# Autodesk Inventor assembly: Jar Jar
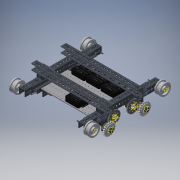
[picture p0: Inventor's stored thumbnail of the model, 180x180]
Saved by Autodesk Inventor 2016 (Build 200138000, 138)
## iProperties
Created: 2015-12-13
Part Number: Jar Jar
Document SubType Name: Assembly
Designer: tbloo
Author: tbloo
## Documents named in this file (16)
- C:\Users\tbloo\Documents\GitHub\phi_robotics\3d-models\FTC_Tetrix_KOP_Block_Party\Tim Bloot Designs\JAr JaR Bot\Jar Jar.iam
- C:\Users\tbloo\Documents\GitHub\phi_robotics\3d-models\FTC_Tetrix_KOP_Block_Party\Tim Bloot Designs\Base Plate.ipt
- C:\Users\tbloo\Documents\GitHub\phi_robotics\3d-models\FTC_Tetrix_KOP_Block_Party\Tetrix_Kit_FTC\Autodesk Inventor Files\tetrix_c_channel-3.ipt
- C:\Users\tbloo\Documents\GitHub\phi_robotics\3d-models\FTC_Tetrix_KOP_Block_Party\Tetrix_Kit_FTC\Autodesk Inventor Files\tetrix_c_channel-2.ipt
- C:\Users\tbloo\Documents\GitHub\phi_robotics\3d-models\FTC_Tetrix_KOP_Block_Party\Tetrix_Kit_FTC\Autodesk Inventor Files\tetrix_motor_mount-old.ipt
- C:\Users\tbloo\Documents\GitHub\phi_robotics\3d-models\FTC_Tetrix_KOP_Block_Party\Tetrix_Kit_FTC\Autodesk Inventor Files\tetrix_739274_2013.ipt
- C:\Users\tbloo\Documents\GitHub\phi_robotics\3d-models\FTC_Tetrix_KOP_Block_Party\Tetrix_Kit_FTC\Autodesk Inventor Files\tetrix_motor.iam
- C:\Users\tbloo\Documents\GitHub\phi_robotics\3d-models\FTC_Tetrix_KOP_Block_Party\Tim Bloot Designs\JAr JaR Bot\Motor Med Gear.iam
- C:\Users\tbloo\Documents\GitHub\phi_robotics\3d-models\FTC_Tetrix_KOP_Block_Party\Tim Bloot Designs\JAr JaR Bot\Tread Sproket Gear Assembly.iam
- C:\Users\tbloo\Documents\GitHub\phi_robotics\3d-models\FTC_Tetrix_KOP_Block_Party\Tetrix_Kit_FTC\Autodesk Inventor Files\tetrix_bushing.ipt
- C:\Users\tbloo\Documents\GitHub\phi_robotics\3d-models\FTC_Tetrix_KOP_Block_Party\Tim Bloot Designs\JAr JaR Bot\Tread Wheel Assembly.iam
- C:\Users\tbloo\Documents\GitHub\phi_robotics\3d-models\FTC_Tetrix_KOP_Block_Party\Tetrix_Kit_FTC\Autodesk Inventor Files\tetrix_angle-144 MM.ipt
- C:\Users\tbloo\Documents\GitHub\phi_robotics\3d-models\FTC_Tetrix_KOP_Block_Party\Tetrix_Kit_FTC\Autodesk Inventor Files\tetrix_c_channel-5.ipt
- C:\Users\tbloo\Documents\GitHub\phi_robotics\3d-models\FTC_Tetrix_KOP_Block_Party\Tetrix_Kit_FTC\Autodesk Inventor Files\tetrix_inside_corner_bracket.ipt
- C:\Users\tbloo\Documents\GitHub\phi_robotics\3d-models\FTC_Tetrix_KOP_Block_Party\Tetrix_Kit_FTC\Autodesk Inventor Files\tetrix_motor_controller.ipt
- C:\Users\tbloo\Documents\GitHub\phi_robotics\3d-models\FTC_Tetrix_KOP_Block_Party\Tetrix_Kit_FTC\Autodesk Inventor Files\tetrix_servo_controller.ipt
## Components (55 placed, 15 different names)
1. Base Plate:1 — Rigid:40, Rigid:53, Rigid:60, Rigid:61, Rigid:63
2. tetrix_c_channel-3:3 — Rigid:37, Rigid:39, Rigid:54, Rigid:57
3. tetrix_c_channel-2:9
4. tetrix_c_channel-2:10
5. tetrix_c_channel-2:11 — Rigid:38
6. tetrix_c_channel-2:12 — Rigid:36
7. tetrix_motor_mount-old:3
8. tetrix_motor_mount-old:4
9. tetrix_739274_2013:3
10. tetrix_739274_2013:4
11. tetrix_motor:3 [sub-assembly]
12. tetrix_motor:4 [sub-assembly]
13. Motor Med Gear:3 [sub-assembly]
14. Motor Med Gear:4 [sub-assembly]
15. Tread Sproket Gear Assembly:3 [sub-assembly]
16. Tread Sproket Gear Assembly:4 [sub-assembly]
17. tetrix_bushing:5
18. tetrix_bushing:6
19. tetrix_bushing:7
20. tetrix_bushing:8
21. Tread Wheel Assembly:3 [sub-assembly]
22. Tread Wheel Assembly:4 [sub-assembly]
23. tetrix_angle-144 MM:1 — Rigid:36, Rigid:37, Rigid:40
24. tetrix_angle-144 MM:2 — Rigid:38, Rigid:39
25. tetrix_c_channel-3:4 — Rigid:55, Rigid:56
26. tetrix_c_channel-2:13
27. tetrix_c_channel-2:14
28. tetrix_c_channel-2:15
29. tetrix_c_channel-2:16
30. tetrix_motor_mount-old:5
31. tetrix_motor_mount-old:6
32. tetrix_739274_2013:5
33. tetrix_739274_2013:6
34. tetrix_motor:5 [sub-assembly]
35. tetrix_motor:6 [sub-assembly]
36. Motor Med Gear:5 [sub-assembly]
37. Motor Med Gear:6 [sub-assembly]
38. Tread Sproket Gear Assembly:5 [sub-assembly]
39. Tread Sproket Gear Assembly:6 [sub-assembly]
40. tetrix_bushing:9
41. tetrix_bushing:10
42. tetrix_bushing:11
43. tetrix_bushing:12
44. Tread Wheel Assembly:5 [sub-assembly]
45. Tread Wheel Assembly:6 [sub-assembly]
46. tetrix_angle-144 MM:3
47. tetrix_angle-144 MM:4 — Rigid:53
48. tetrix_c_channel-5:1 — Rigid:54, Rigid:55
49. tetrix_c_channel-5:2 — Rigid:58, Rigid:59
50. tetrix_inside_corner_bracket:1 — Rigid:57, Rigid:58
51. tetrix_inside_corner_bracket:2 — Rigid:56, Rigid:59
52. tetrix_motor_controller:1 — Rigid:61, Rigid:62
53. tetrix_motor_controller:2 — Rigid:60
54. tetrix_motor_controller:3 — Rigid:62
55. tetrix_servo_controller:1 — Rigid:63
## Relationships (56: WeldJoint 36, RevoluteJoint 20)
- [WeldJoint]: tetrix_c_channel-2:9 ↔ tetrix_motor_mount-old:4
- [WeldJoint]: tetrix_c_channel-2:10 ↔ tetrix_motor_mount-old:3
- [WeldJoint]: tetrix_c_channel-2:9 ↔ tetrix_739274_2013:3
- [WeldJoint]: tetrix_c_channel-2:11 ↔ tetrix_739274_2013:3
- [WeldJoint]: tetrix_c_channel-2:10 ↔ tetrix_739274_2013:4
- [WeldJoint]: tetrix_c_channel-2:12 ↔ tetrix_739274_2013:4
- [RevoluteJoint]: tetrix_motor_mount-old:4 ↔ tetrix_motor:3
- [RevoluteJoint]: tetrix_motor_mount-old:3 ↔ tetrix_motor:4
- [WeldJoint] (-7.5 mm): tetrix_motor:4 ↔ Motor Med Gear:3
- [WeldJoint] (-7.5 mm): tetrix_motor:3 ↔ Motor Med Gear:4
- [RevoluteJoint]: tetrix_c_channel-2:9 ↔ tetrix_bushing:6
- [RevoluteJoint]: tetrix_c_channel-2:9 ↔ tetrix_bushing:5
- [RevoluteJoint]: Tread Sproket Gear Assembly:3 ↔ tetrix_bushing:5
- [RevoluteJoint]: tetrix_c_channel-2:10 ↔ tetrix_bushing:7
- [RevoluteJoint]: tetrix_c_channel-2:10 ↔ tetrix_bushing:8
- [RevoluteJoint]: Tread Sproket Gear Assembly:4 ↔ tetrix_bushing:8
- [RevoluteJoint]: tetrix_c_channel-2:11 ↔ Tread Wheel Assembly:3
- [RevoluteJoint]: tetrix_c_channel-2:12 ↔ Tread Wheel Assembly:4
- Rigid:36 [WeldJoint]: tetrix_c_channel-2:12 ↔ tetrix_angle-144 MM:1
- Rigid:37 [WeldJoint]: tetrix_c_channel-3:3 ↔ tetrix_angle-144 MM:1
- Rigid:38 [WeldJoint]: tetrix_c_channel-2:11 ↔ tetrix_angle-144 MM:2
- Rigid:39 [WeldJoint]: tetrix_c_channel-3:3 ↔ tetrix_angle-144 MM:2
- Rigid:40 [WeldJoint]: Base Plate:1 ↔ tetrix_angle-144 MM:1
- [WeldJoint]: tetrix_c_channel-2:13 ↔ tetrix_motor_mount-old:6
- [WeldJoint]: tetrix_c_channel-2:14 ↔ tetrix_motor_mount-old:5
- [WeldJoint]: tetrix_c_channel-2:13 ↔ tetrix_739274_2013:5
- [WeldJoint]: tetrix_c_channel-2:15 ↔ tetrix_739274_2013:5
- [WeldJoint]: tetrix_c_channel-2:14 ↔ tetrix_739274_2013:6
- [WeldJoint]: tetrix_c_channel-2:16 ↔ tetrix_739274_2013:6
- [RevoluteJoint]: tetrix_motor_mount-old:6 ↔ tetrix_motor:5
- [RevoluteJoint]: tetrix_motor_mount-old:5 ↔ tetrix_motor:6
- [WeldJoint] (-7.5 mm): tetrix_motor:6 ↔ Motor Med Gear:5
- [WeldJoint] (-7.5 mm): tetrix_motor:5 ↔ Motor Med Gear:6
- [RevoluteJoint]: tetrix_c_channel-2:13 ↔ tetrix_bushing:10
- [RevoluteJoint]: tetrix_c_channel-2:13 ↔ tetrix_bushing:9
- [RevoluteJoint]: Tread Sproket Gear Assembly:5 ↔ tetrix_bushing:9
- [RevoluteJoint]: tetrix_c_channel-2:14 ↔ tetrix_bushing:11
- [RevoluteJoint]: tetrix_c_channel-2:14 ↔ tetrix_bushing:12
- [RevoluteJoint]: Tread Sproket Gear Assembly:6 ↔ tetrix_bushing:12
- [RevoluteJoint]: tetrix_c_channel-2:15 ↔ Tread Wheel Assembly:5
- [RevoluteJoint]: tetrix_c_channel-2:16 ↔ Tread Wheel Assembly:6
- [WeldJoint]: tetrix_c_channel-2:16 ↔ tetrix_angle-144 MM:3
- [WeldJoint]: tetrix_c_channel-3:4 ↔ tetrix_angle-144 MM:3
- [WeldJoint]: tetrix_c_channel-2:15 ↔ tetrix_angle-144 MM:4
- [WeldJoint]: tetrix_c_channel-3:4 ↔ tetrix_angle-144 MM:4
- Rigid:53 [WeldJoint]: Base Plate:1 ↔ tetrix_angle-144 MM:4
- Rigid:54 [WeldJoint]: tetrix_c_channel-3:3 ↔ tetrix_c_channel-5:1
- Rigid:55 [WeldJoint]: tetrix_c_channel-3:4 ↔ tetrix_c_channel-5:1
- Rigid:56 [WeldJoint]: tetrix_c_channel-3:4 ↔ tetrix_inside_corner_bracket:2
- Rigid:57 [WeldJoint]: tetrix_c_channel-3:3 ↔ tetrix_inside_corner_bracket:1
- Rigid:58 [WeldJoint]: tetrix_c_channel-5:2 ↔ tetrix_inside_corner_bracket:1
- Rigid:59 [WeldJoint]: tetrix_c_channel-5:2 ↔ tetrix_inside_corner_bracket:2
- Rigid:60 [WeldJoint]: Base Plate:1 ↔ tetrix_motor_controller:2
- Rigid:61 [WeldJoint]: Base Plate:1 ↔ tetrix_motor_controller:1
- Rigid:62 [WeldJoint]: tetrix_motor_controller:1 ↔ tetrix_motor_controller:3
- Rigid:63 [WeldJoint]: Base Plate:1 ↔ tetrix_servo_controller:1
## Named parameters: d44_d25 = -7.5 mm, d45_d26 = -7.5 mm, d46_d27 = 0 mm, d47_d28 = 4.697383 deg, d48_d29 = 0 mm, d49_d30 = 0.338188 deg, d50_d31 = 0 mm, d51_d32 = -0.013892 deg, d52_d33 = 0 mm, d53_d34 = 0.814021 deg, d54_d35 = 0 mm, d55_d36 = -29.078357 deg, d56_d37 = 0 mm, d57_d38 = 29.910319 deg, d58_d39 = 0 mm, d59_d40 = -5.431137 deg, d60_d41 = 0 mm, d61_d42 = 0.840635 deg, d65_d11 = 0 mm, d66_d12 = 0 mm, d67_d13 = 0 mm, d68_d14 = 0 mm, d69_d15 = 0 mm, d70_d16 = 0 mm, d71_d21 = 0 mm, d72_d22 = -9.167541 deg, d73_d23 = 0 mm, d74_d24 = -19.058032 deg, d94_d89 = 0 mm, d95_d90 = 0 mm, d96_d91 = 0 mm, d97_d92 = 0 mm, d98_d44_d25 = -7.5 mm, d99_d45_d26 = -7.5 mm, d100_d46_d27 = 0 mm, d101_d47_d28 = 4.697383 deg, d102_d48_d29 = 0 mm, d103_d49_d30 = 0.338188 deg, d104_d50_d31 = 0 mm, d105_d51_d32 = -0.013892 deg, d106_d52_d33 = 0 mm, d107_d53_d34 = 0.814021 deg, d108_d54_d35 = 0 mm, d109_d55_d36 = -29.078357 deg, d110_d56_d37 = 0 mm, d111_d57_d38 = 29.910319 deg, d112_d58_d39 = 0 mm, d113_d59_d40 = -5.431137 deg, d114_d60_d41 = 0 mm, d115_d61_d42 = 0.840635 deg, d116_d65_d11 = 0 mm, d117_d66_d12 = 0 mm, d118_d67_d13 = 0 mm, d119_d68_d14 = 0 mm, d120_d69_d15 = 0 mm, d121_d70_d16 = 0 mm, d122_d71_d21 = 0 mm, d123_d72_d22 = -45.624239 deg, d124_d73_d23 = 0 mm, d125_d74_d24 = -134.077368 deg
